# Autodesk Inventor assembly: Switch Assembly
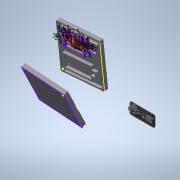
[picture p0: Inventor's stored thumbnail of the model, 180x180]
Saved by Autodesk Inventor 2020.2 (Build 242310000, 310)
## iProperties
Created: 2019-11-25
Part Number: Switch Assembly
Document SubType Name: Assembly
Designer: Administrator
Title: WICED Feather v12 v1
Author: Administrator
## Documents named in this file (17)
- C:\Users\athiy\OneDrive\S2\01 KULIAH\SURG0094 Group Research Project\3D drawing\Switch Assembly.iam
- C:\Users\athiy\OneDrive\S2\01 KULIAH\SURG0094 Group Research Project\3D drawing\WICED Feather v12 v1\board.ipt
- C:\Users\athiy\OneDrive\S2\01 KULIAH\SURG0094 Group Research Project\3D drawing\WICED Feather v12 v1\P0.ipt
- C:\Users\athiy\OneDrive\S2\01 KULIAH\SURG0094 Group Research Project\3D drawing\WICED Feather v12 v1\P0 solder.ipt
- C:\Users\athiy\OneDrive\S2\01 KULIAH\SURG0094 Group Research Project\3D drawing\WICED Feather v12 v1\jst_2_adafruit_1769 v2.iam
- C:\Users\athiy\OneDrive\S2\01 KULIAH\SURG0094 Group Research Project\3D drawing\WICED Feather v12 v1\TSOP-5 v3.ipt
- C:\Users\athiy\OneDrive\S2\01 KULIAH\SURG0094 Group Research Project\3D drawing\WICED Feather v12 v1\cap0805_05 v2.ipt
- C:\Users\athiy\OneDrive\S2\01 KULIAH\SURG0094 Group Research Project\3D drawing\WICED Feather v12 v1\cap0805_03 v2.ipt
- C:\Users\athiy\OneDrive\S2\01 KULIAH\SURG0094 Group Research Project\3D drawing\WICED Feather v12 v1\cap0603_03 v3.ipt
- C:\Users\athiy\OneDrive\S2\01 KULIAH\SURG0094 Group Research Project\3D drawing\WICED Feather v12 v1\smt_tact_button v3.ipt
- C:\Users\athiy\OneDrive\S2\01 KULIAH\SURG0094 Group Research Project\3D drawing\WICED Feather v12 v1\micro_usb_47346-0001 v2.iam
- C:\Users\athiy\OneDrive\S2\01 KULIAH\SURG0094 Group Research Project\3D drawing\WICED Feather v12 v1\resistor_0603 v2.ipt
- C:\Users\athiy\OneDrive\S2\01 KULIAH\SURG0094 Group Research Project\3D drawing\WICED Feather v12 v1\sioc-8 v5.iam
- C:\Users\athiy\OneDrive\S2\01 KULIAH\SURG0094 Group Research Project\3D drawing\WICED Feather v12 v1\smt_led_0805 v2.ipt
- C:\Users\athiy\OneDrive\S2\01 KULIAH\SURG0094 Group Research Project\3D drawing\WICED Feather v12 v1\Voice Recognition Module-01.ipt
- C:\Users\athiy\OneDrive\S2\01 KULIAH\SURG0094 Group Research Project\3D drawing\Case rev.0.ipt
- C:\Users\athiy\OneDrive\S2\01 KULIAH\SURG0094 Group Research Project\3D drawing\Case Cover rev.0.ipt
## Components (29 placed, 16 different names)
1. board:1
2. P0:1
3. P0 solder:1
4. jst_2_adafruit_1769 v2:1 [sub-assembly]
5. TSOP-5 v3:1
6. TSOP-5 v3:2
7. cap0805_05 v2:1
8. cap0805_03 v2:1
9. cap0603_03 v3:1
10. smt_tact_button v3:1
11. micro_usb_47346-0001 v2:1 [sub-assembly]
12. cap0603_03 v3:2
13. cap0805_05 v2:2
14. cap0805_05 v2:3
15. cap0805_05 v2:4
16. cap0805_05 v2:5
17. resistor_0603 v2:1
18. sioc-8 v5:1 [sub-assembly]
19. smt_led_0805 v2:1
20. resistor_0603 v2:2
21. resistor_0603 v2:3
22. resistor_0603 v2:4
23. resistor_0603 v2:5
24. resistor_0603 v2:6
25. resistor_0603 v2:7
26. smt_led_0805 v2:2
27. Voice Recognition Module-01:1 — Mate:1, Mate:2
28. Case rev.0:1 — Mate:1, Mate:2
29. Case Cover rev.0:1
## Relationships (2: Mate 2)
- Mate:1: Voice Recognition Module-01:1 ↔ Case rev.0:1
- Mate:2: Voice Recognition Module-01:1 ↔ Case rev.0:1
